# Autodesk Inventor assembly: am-3448 PicoBox Duo REV2
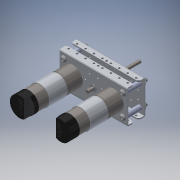
[picture p0: Inventor's stored thumbnail of the model, 180x180]
Saved by Autodesk Inventor 2019 (Build 230136000, 136)
## iProperties
Created: 2018-06-18
Part Number: am-3448 PicoBox Duo REV2
Description: STEP AP214
Document SubType Name: Assembly
Designer: james
Sending System: SolidWorks 2017
Preprocessor: SwSTEP 2.0
Title: am-3448 PicoBox Duo REV2.STEP
Revision Number: ANY
## Documents named in this file (15)
- F:\JimsDesign\Library\AndyMark\am-3448 PicoBox Duo REV2.iam
- F:\JimsDesign\Library\AndyMark\PicoBox Duo Plate.ipt
- F:\JimsDesign\Library\AndyMark\PicoBox Spacer.ipt
- F:\JimsDesign\Library\AndyMark\6mm x 12mm Flanged -Mcm 7804K142_7804K142.ipt
- F:\JimsDesign\Library\AndyMark\am-2964 NeveRest.ipt
- F:\JimsDesign\Library\AndyMark\am-3215 6mmD Double Boss Nub.ipt
- F:\JimsDesign\Library\AndyMark\40T 32DP 20PA With 6mm Bore Nub Gear.ipt
- F:\JimsDesign\Library\AndyMark\14-20 x 1.750 BHCS_92949A837.ipt
- F:\JimsDesign\Library\AndyMark\14-20 NyLock thin - Mcm 90566A029_90566A029.ipt
- F:\JimsDesign\Library\AndyMark\M3x0.5x6mm SHCS_91290A111.ipt
- F:\JimsDesign\Library\AndyMark\6-32 x 0500 HHCS_93075A148.ipt
- F:\JimsDesign\Library\AndyMark\10-32 x 0.25 Set Screw Cup Point.ipt
- F:\JimsDesign\Library\AndyMark\6mm D-Shaft 100mm.ipt
- F:\JimsDesign\Library\AndyMark\PicoBoxOutsideSpacers.ipt
- F:\JimsDesign\Library\AndyMark\PicoBoxInsideSpacers.ipt
## Components (58 placed, 55 different names)
1. PicoBox Duo Plate_1 — Mate:1, Mate:2, Mate:3, Mate:4, Mate:5, Mate:6, Mate:7, Mate:8, Mate:9, Mate:10, Mate:11, Mate:12, Mate:13, Mate:14, Mate:15, Mate:16, Mate:17, Mate:18, Mate:19, Mate:20, Mate:21, Mate:22, Mate:23, Mate:24, Mate:25, Mate:26, Mate:27, Mate:28, Mate:31, Mate:32, Mate:33, Mate:34, Mate:35, Mate:36, Mate:37, Mate:38, Mate:39, Mate:40, Mate:41, Mate:43, Mate:45, Mate:47
2. PicoBox Spacer_2 — Mate:41, Mate:42
3. PicoBox Spacer_3 — Mate:45, Mate:46, Mate:64
4. PicoBox Spacer_4 — Mate:47, Mate:48, Mate:62, Mate:63
5. PicoBox Spacer_5 — Mate:43, Mate:44
6. 6mm x 12mm Flanged -Mcm 7804K142_7804K142_6 — Mate:39, Mate:40, Mate:106
7. am-2964 NeveRest_7 — Mate:26, Mate:27, Mate:29, Mate:60, Mate:61, Mate:110
8. am-2964 NeveRest_8 — Mate:25, Mate:28, Mate:30, Mate:92, Mate:93, Mate:109
9. am-3215 6mmD Double Boss Nub_9 — Mate:49, Mate:50, Mate:55, Mate:61, Mate:65, Mate:111
10. am-3215 6mmD Double Boss Nub_10 — Mate:102, Mate:103, Mate:104, Mate:105, Mate:107, Mate:112
11. am-3215 6mmD Double Boss Nub_11 — Mate:80, Mate:81, Mate:82, Mate:91, Mate:93, Mate:108
12. 6mm x 12mm Flanged -Mcm 7804K142_7804K142_12 — Mate:74, Mate:75
13. 40T 32DP 20PA With 6mm Bore Nub Gear_13 — Mate:49, Mate:50, Mate:51, Mate:52, Mate:53, Mate:54, Mate:56, Mate:57, Mate:58, Mate:59, Mate:60, Flush:1
14. 40T 32DP 20PA With 6mm Bore Nub Gear_14 — Mate:94, Mate:95, Mate:96, Mate:97, Mate:98, Mate:99, Mate:100, Mate:101, Mate:102, Mate:104, Flush:1, Mate:114
15. 40T 32DP 20PA With 6mm Bore Nub Gear_15 — Mate:80, Mate:81, Mate:82, Mate:83, Mate:84, Mate:85, Mate:86, Mate:87, Mate:88, Mate:89, Mate:90, Mate:92
16. 14-20 x 1.750 BHCS_92949A837_16 — Mate:31, Mate:38, Mate:44, Mate:69
17. 14-20 x 1.750 BHCS_92949A837_17 — Mate:32, Mate:37, Mate:42, Mate:73
18. 14-20 x 1.750 BHCS_92949A837_18 — Mate:34, Mate:35, Mate:48, Mate:71
19. 14-20 x 1.750 BHCS_92949A837_19 — Mate:33, Mate:36, Mate:46, Mate:67
20. 14-20 NyLock thin - Mcm 90566A029_90566A029_20 — Mate:66, Mate:67
21. 14-20 NyLock thin - Mcm 90566A029_90566A029_21 — Mate:72, Mate:73
22. 14-20 NyLock thin - Mcm 90566A029_90566A029_22 — Mate:70, Mate:71
23. 14-20 NyLock thin - Mcm 90566A029_90566A029_23 — Mate:68, Mate:69
24. M3x0.5x6mm SHCS_91290A111_24 — Mate:8, Mate:21
25. M3x0.5x6mm SHCS_91290A111_25 — Mate:2, Mate:23
26. M3x0.5x6mm SHCS_91290A111_26 — Mate:4, Mate:22
27. M3x0.5x6mm SHCS_91290A111_27 — Mate:9, Mate:16
28. M3x0.5x6mm SHCS_91290A111_28 — Mate:10, Mate:15, Mate:29
29. M3x0.5x6mm SHCS_91290A111_29 — Mate:3, Mate:18
30. M3x0.5x6mm SHCS_91290A111_30 — Mate:7, Mate:17
31. M3x0.5x6mm SHCS_91290A111_31 — Mate:5, Mate:24
32. M3x0.5x6mm SHCS_91290A111_32 — Mate:1, Mate:13
33. M3x0.5x6mm SHCS_91290A111_33 — Mate:12, Mate:20
34. M3x0.5x6mm SHCS_91290A111_34 — Mate:6, Mate:19, Mate:30
35. M3x0.5x6mm SHCS_91290A111_35 — Mate:11, Mate:14
36. 6-32 x 0500 HHCS_93075A148_36 — Mate:51, Mate:53
37. 6-32 x 0500 HHCS_93075A148_37 — Mate:84, Mate:87
38. 6-32 x 0500 HHCS_93075A148_38 — Mate:100, Mate:101
39. 6-32 x 0500 HHCS_93075A148_39 — Mate:57, Mate:58
40. 6-32 x 0500 HHCS_93075A148_40 — Mate:52, Mate:54, Mate:55
41. 6-32 x 0500 HHCS_93075A148_41 — Mate:56, Mate:59
42. 6-32 x 0500 HHCS_93075A148_42 — Mate:85, Mate:88
43. 6-32 x 0500 HHCS_93075A148_43 — Mate:96, Mate:99, Mate:105
44. 6-32 x 0500 HHCS_93075A148_44 — Mate:94, Mate:97
45. 6-32 x 0500 HHCS_93075A148_45 — Mate:83, Mate:86
46. 6-32 x 0500 HHCS_93075A148_46 — Mate:89, Mate:90
47. 6-32 x 0500 HHCS_93075A148_47 — Mate:95, Mate:98
48. 10-32 x 0.25 Set Screw Cup Point_48 — Mate:103
49. 10-32 x 0.25 Set Screw Cup Point_49 — Mate:91
50. 10-32 x 0.25 Set Screw Cup Point_50 — Mate:65
51. PicoBox Duo Plate_51 — Mate:62, Mate:63, Mate:64, Mate:66, Mate:68, Mate:70, Mate:72, Mate:74, Mate:75, Mate:76, Mate:77, Mate:78, Mate:79
52. 6mm D-Shaft 100mm_52 — Mate:106, Mate:107, Mate:113, Mate:115
53. 6mm x 12mm Flanged -Mcm 7804K142_7804K142:3 — Mate:76, Mate:77
54. 6mm x 12mm Flanged -Mcm 7804K142_7804K142:4 — Mate:78, Mate:79
55. PicoBoxOutsideSpacers:1 — Mate:108, Mate:109
56. PicoBoxOutsideSpacers:2 — Mate:110, Mate:111
57. PicoBoxOutsideSpacers:3 — Mate:112, Mate:113
58. PicoBoxInsideSpacers:1 — Mate:114, Mate:115
## Relationships (116: Mate 115, Flush 1)
- Mate:1: PicoBox Duo Plate_1 ↔ M3x0.5x6mm SHCS_91290A111_32
- Mate:2: PicoBox Duo Plate_1 ↔ M3x0.5x6mm SHCS_91290A111_25
- Mate:3: PicoBox Duo Plate_1 ↔ M3x0.5x6mm SHCS_91290A111_29
- Mate:4: PicoBox Duo Plate_1 ↔ M3x0.5x6mm SHCS_91290A111_26
- Mate:5: PicoBox Duo Plate_1 ↔ M3x0.5x6mm SHCS_91290A111_31
- Mate:6: PicoBox Duo Plate_1 ↔ M3x0.5x6mm SHCS_91290A111_34
- Mate:7: PicoBox Duo Plate_1 ↔ M3x0.5x6mm SHCS_91290A111_30
- Mate:8: PicoBox Duo Plate_1 ↔ M3x0.5x6mm SHCS_91290A111_24
- Mate:9: PicoBox Duo Plate_1 ↔ M3x0.5x6mm SHCS_91290A111_27
- Mate:10: PicoBox Duo Plate_1 ↔ M3x0.5x6mm SHCS_91290A111_28
- Mate:11: PicoBox Duo Plate_1 ↔ M3x0.5x6mm SHCS_91290A111_35
- Mate:12: PicoBox Duo Plate_1 ↔ M3x0.5x6mm SHCS_91290A111_33
- Mate:13: PicoBox Duo Plate_1 ↔ M3x0.5x6mm SHCS_91290A111_32
- Mate:14: PicoBox Duo Plate_1 ↔ M3x0.5x6mm SHCS_91290A111_35
- Mate:15: PicoBox Duo Plate_1 ↔ M3x0.5x6mm SHCS_91290A111_28
- Mate:16: PicoBox Duo Plate_1 ↔ M3x0.5x6mm SHCS_91290A111_27
- Mate:17: PicoBox Duo Plate_1 ↔ M3x0.5x6mm SHCS_91290A111_30
- Mate:18: PicoBox Duo Plate_1 ↔ M3x0.5x6mm SHCS_91290A111_29
- Mate:19: PicoBox Duo Plate_1 ↔ M3x0.5x6mm SHCS_91290A111_34
- Mate:20: PicoBox Duo Plate_1 ↔ M3x0.5x6mm SHCS_91290A111_33
- Mate:21: PicoBox Duo Plate_1 ↔ M3x0.5x6mm SHCS_91290A111_24
- Mate:22: PicoBox Duo Plate_1 ↔ M3x0.5x6mm SHCS_91290A111_26
- Mate:23: PicoBox Duo Plate_1 ↔ M3x0.5x6mm SHCS_91290A111_25
- Mate:24: PicoBox Duo Plate_1 ↔ M3x0.5x6mm SHCS_91290A111_31
- Mate:25: PicoBox Duo Plate_1 ↔ am-2964 NeveRest_8
- Mate:26: PicoBox Duo Plate_1 ↔ am-2964 NeveRest_7
- Mate:27: PicoBox Duo Plate_1 ↔ am-2964 NeveRest_7
- Mate:28: PicoBox Duo Plate_1 ↔ am-2964 NeveRest_8
- Mate:29: am-2964 NeveRest_7 ↔ M3x0.5x6mm SHCS_91290A111_28
- Mate:30: am-2964 NeveRest_8 ↔ M3x0.5x6mm SHCS_91290A111_34
- Mate:31: PicoBox Duo Plate_1 ↔ 14-20 x 1.750 BHCS_92949A837_16
- Mate:32: PicoBox Duo Plate_1 ↔ 14-20 x 1.750 BHCS_92949A837_17
- Mate:33: PicoBox Duo Plate_1 ↔ 14-20 x 1.750 BHCS_92949A837_19
- Mate:34: PicoBox Duo Plate_1 ↔ 14-20 x 1.750 BHCS_92949A837_18
- Mate:35: PicoBox Duo Plate_1 ↔ 14-20 x 1.750 BHCS_92949A837_18
- Mate:36: PicoBox Duo Plate_1 ↔ 14-20 x 1.750 BHCS_92949A837_19
- Mate:37: PicoBox Duo Plate_1 ↔ 14-20 x 1.750 BHCS_92949A837_17
- Mate:38: PicoBox Duo Plate_1 ↔ 14-20 x 1.750 BHCS_92949A837_16
- Mate:39: PicoBox Duo Plate_1 ↔ 6mm x 12mm Flanged -Mcm 7804K142_7804K142_6
- Mate:40: PicoBox Duo Plate_1 ↔ 6mm x 12mm Flanged -Mcm 7804K142_7804K142_6
- Mate:41: PicoBox Duo Plate_1 ↔ PicoBox Spacer_2
- Mate:42: PicoBox Spacer_2 ↔ 14-20 x 1.750 BHCS_92949A837_17
- Mate:43: PicoBox Duo Plate_1 ↔ PicoBox Spacer_5
- Mate:44: PicoBox Spacer_5 ↔ 14-20 x 1.750 BHCS_92949A837_16
- Mate:45: PicoBox Duo Plate_1 ↔ PicoBox Spacer_3
- Mate:46: PicoBox Spacer_3 ↔ 14-20 x 1.750 BHCS_92949A837_19
- Mate:47: PicoBox Duo Plate_1 ↔ PicoBox Spacer_4
- Mate:48: PicoBox Spacer_4 ↔ 14-20 x 1.750 BHCS_92949A837_18
- Mate:49: am-3215 6mmD Double Boss Nub_9 ↔ 40T 32DP 20PA With 6mm Bore Nub Gear_13
- Mate:50: am-3215 6mmD Double Boss Nub_9 ↔ 40T 32DP 20PA With 6mm Bore Nub Gear_13
- Mate:51: 40T 32DP 20PA With 6mm Bore Nub Gear_13 ↔ 6-32 x 0500 HHCS_93075A148_36
- Mate:52: 40T 32DP 20PA With 6mm Bore Nub Gear_13 ↔ 6-32 x 0500 HHCS_93075A148_40
- Mate:53: 40T 32DP 20PA With 6mm Bore Nub Gear_13 ↔ 6-32 x 0500 HHCS_93075A148_36
- Mate:54: 40T 32DP 20PA With 6mm Bore Nub Gear_13 ↔ 6-32 x 0500 HHCS_93075A148_40
- Mate:55: am-3215 6mmD Double Boss Nub_9 ↔ 6-32 x 0500 HHCS_93075A148_40
- Mate:56: 40T 32DP 20PA With 6mm Bore Nub Gear_13 ↔ 6-32 x 0500 HHCS_93075A148_41
- Mate:57: 40T 32DP 20PA With 6mm Bore Nub Gear_13 ↔ 6-32 x 0500 HHCS_93075A148_39
- Mate:58: 40T 32DP 20PA With 6mm Bore Nub Gear_13 ↔ 6-32 x 0500 HHCS_93075A148_39
- Mate:59: 40T 32DP 20PA With 6mm Bore Nub Gear_13 ↔ 6-32 x 0500 HHCS_93075A148_41
- Mate:60: am-2964 NeveRest_7 ↔ 40T 32DP 20PA With 6mm Bore Nub Gear_13
- Mate:61: am-2964 NeveRest_7 ↔ am-3215 6mmD Double Boss Nub_9
- Mate:62: PicoBox Spacer_4 ↔ PicoBox Duo Plate_51
- Mate:63: PicoBox Spacer_4 ↔ PicoBox Duo Plate_51
- Mate:64: PicoBox Spacer_3 ↔ PicoBox Duo Plate_51
- Mate:65: am-3215 6mmD Double Boss Nub_9 ↔ 10-32 x 0.25 Set Screw Cup Point_50
- Mate:66: 14-20 NyLock thin - Mcm 90566A029_90566A029_20 ↔ PicoBox Duo Plate_51
- Mate:67: 14-20 x 1.750 BHCS_92949A837_19 ↔ 14-20 NyLock thin - Mcm 90566A029_90566A029_20
- Mate:68: 14-20 NyLock thin - Mcm 90566A029_90566A029_23 ↔ PicoBox Duo Plate_51
- Mate:69: 14-20 x 1.750 BHCS_92949A837_16 ↔ 14-20 NyLock thin - Mcm 90566A029_90566A029_23
- Mate:70: 14-20 NyLock thin - Mcm 90566A029_90566A029_22 ↔ PicoBox Duo Plate_51
- Mate:71: 14-20 x 1.750 BHCS_92949A837_18 ↔ 14-20 NyLock thin - Mcm 90566A029_90566A029_22
- Mate:72: 14-20 NyLock thin - Mcm 90566A029_90566A029_21 ↔ PicoBox Duo Plate_51
- Mate:73: 14-20 x 1.750 BHCS_92949A837_17 ↔ 14-20 NyLock thin - Mcm 90566A029_90566A029_21
- Mate:74: 6mm x 12mm Flanged -Mcm 7804K142_7804K142_12 ↔ PicoBox Duo Plate_51
- Mate:75: 6mm x 12mm Flanged -Mcm 7804K142_7804K142_12 ↔ PicoBox Duo Plate_51
- Mate:76: PicoBox Duo Plate_51 ↔ 6mm x 12mm Flanged -Mcm 7804K142_7804K142:3
- Mate:77: PicoBox Duo Plate_51 ↔ 6mm x 12mm Flanged -Mcm 7804K142_7804K142:3
- Mate:78: PicoBox Duo Plate_51 ↔ 6mm x 12mm Flanged -Mcm 7804K142_7804K142:4
- Mate:79: PicoBox Duo Plate_51 ↔ 6mm x 12mm Flanged -Mcm 7804K142_7804K142:4
- Mate:80: am-3215 6mmD Double Boss Nub_11 ↔ 40T 32DP 20PA With 6mm Bore Nub Gear_15
- Mate:81: am-3215 6mmD Double Boss Nub_11 ↔ 40T 32DP 20PA With 6mm Bore Nub Gear_15
- Mate:82: am-3215 6mmD Double Boss Nub_11 ↔ 40T 32DP 20PA With 6mm Bore Nub Gear_15
- Mate:83: 40T 32DP 20PA With 6mm Bore Nub Gear_15 ↔ 6-32 x 0500 HHCS_93075A148_45
- Mate:84: 40T 32DP 20PA With 6mm Bore Nub Gear_15 ↔ 6-32 x 0500 HHCS_93075A148_37
- Mate:85: 40T 32DP 20PA With 6mm Bore Nub Gear_15 ↔ 6-32 x 0500 HHCS_93075A148_42
- Mate:86: 40T 32DP 20PA With 6mm Bore Nub Gear_15 ↔ 6-32 x 0500 HHCS_93075A148_45
- Mate:87: 40T 32DP 20PA With 6mm Bore Nub Gear_15 ↔ 6-32 x 0500 HHCS_93075A148_37
- Mate:88: 40T 32DP 20PA With 6mm Bore Nub Gear_15 ↔ 6-32 x 0500 HHCS_93075A148_42
- Mate:89: 40T 32DP 20PA With 6mm Bore Nub Gear_15 ↔ 6-32 x 0500 HHCS_93075A148_46
- Mate:90: 40T 32DP 20PA With 6mm Bore Nub Gear_15 ↔ 6-32 x 0500 HHCS_93075A148_46
- Mate:91: am-3215 6mmD Double Boss Nub_11 ↔ 10-32 x 0.25 Set Screw Cup Point_49
- Mate:92: am-2964 NeveRest_8 ↔ 40T 32DP 20PA With 6mm Bore Nub Gear_15
- Mate:93: am-2964 NeveRest_8 ↔ am-3215 6mmD Double Boss Nub_11
- Mate:94: 40T 32DP 20PA With 6mm Bore Nub Gear_14 ↔ 6-32 x 0500 HHCS_93075A148_44
- Mate:95: 40T 32DP 20PA With 6mm Bore Nub Gear_14 ↔ 6-32 x 0500 HHCS_93075A148_47
- Mate:96: 40T 32DP 20PA With 6mm Bore Nub Gear_14 ↔ 6-32 x 0500 HHCS_93075A148_43
- Mate:97: 40T 32DP 20PA With 6mm Bore Nub Gear_14 ↔ 6-32 x 0500 HHCS_93075A148_44
- Mate:98: 40T 32DP 20PA With 6mm Bore Nub Gear_14 ↔ 6-32 x 0500 HHCS_93075A148_47
- Mate:99: 40T 32DP 20PA With 6mm Bore Nub Gear_14 ↔ 6-32 x 0500 HHCS_93075A148_43
- Mate:100: 40T 32DP 20PA With 6mm Bore Nub Gear_14 ↔ 6-32 x 0500 HHCS_93075A148_38
- Mate:101: 40T 32DP 20PA With 6mm Bore Nub Gear_14 ↔ 6-32 x 0500 HHCS_93075A148_38
- Mate:102: am-3215 6mmD Double Boss Nub_10 ↔ 40T 32DP 20PA With 6mm Bore Nub Gear_14
- Mate:103: am-3215 6mmD Double Boss Nub_10 ↔ 10-32 x 0.25 Set Screw Cup Point_48
- Mate:104: am-3215 6mmD Double Boss Nub_10 ↔ 40T 32DP 20PA With 6mm Bore Nub Gear_14
- Mate:105: am-3215 6mmD Double Boss Nub_10 ↔ 6-32 x 0500 HHCS_93075A148_43
- Mate:106: 6mm x 12mm Flanged -Mcm 7804K142_7804K142_6 ↔ 6mm D-Shaft 100mm_52
- Flush:1: 40T 32DP 20PA With 6mm Bore Nub Gear_13 ↔ 40T 32DP 20PA With 6mm Bore Nub Gear_14
- Mate:107: am-3215 6mmD Double Boss Nub_10 ↔ 6mm D-Shaft 100mm_52
- Mate:108: am-3215 6mmD Double Boss Nub_11 ↔ PicoBoxOutsideSpacers:1
- Mate:109: am-2964 NeveRest_8 ↔ PicoBoxOutsideSpacers:1
- Mate:110: am-2964 NeveRest_7 ↔ PicoBoxOutsideSpacers:2
- Mate:111: am-3215 6mmD Double Boss Nub_9 ↔ PicoBoxOutsideSpacers:2
- Mate:112: am-3215 6mmD Double Boss Nub_10 ↔ PicoBoxOutsideSpacers:3
- Mate:113: 6mm D-Shaft 100mm_52 ↔ PicoBoxOutsideSpacers:3
- Mate:114: 40T 32DP 20PA With 6mm Bore Nub Gear_14 ↔ PicoBoxInsideSpacers:1
- Mate:115: 6mm D-Shaft 100mm_52 ↔ PicoBoxInsideSpacers:1
